# Autodesk Inventor assembly: 69. Блок шестерен промежуточного вала
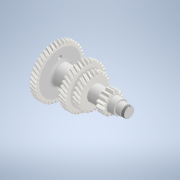
[picture p0: Inventor's stored thumbnail of the model, 180x180]
Saved by Autodesk Inventor 2021 (Build 250183000, 183)
## iProperties
Created: 2021-03-22
Part Number: 69. Блок шестерен промежуточного вала
Document SubType Name: Assembly
Designer: Данил
Author: Данил
## Documents named in this file (6)
- C:\Users\Данил\Desktop\Коробка передач\Детали\69. Блок шестерен промежуточного вала.iam
- C:\Users\Данил\Desktop\Коробка передач\Детали\69. Блок шестерен промежуточного вала.ipt
- C:\Users\Данил\Desktop\Коробка передач\Детали\69. Блок шестерен промежуточного вала\Мастер проектирования\Цилиндрическое зубчатое зацепление1.iam
- C:\Users\Данил\Desktop\Коробка передач\Детали\69. Блок шестерен промежуточного вала\Мастер проектирования\Цилиндрическое зубчатое зацепление2.iam
- C:\Users\Данил\Desktop\Коробка передач\Детали\69. Блок шестерен промежуточного вала\Мастер проектирования\Цилиндрическое зубчатое зацепление3.iam
- C:\Users\Данил\Desktop\Коробка передач\Детали\69. Блок шестерен промежуточного вала\Мастер проектирования\Цилиндрическое зубчатое зацепление4.iam
## Components (5 placed, 2 different names)
1. 69. Блок шестерен промежуточного вала:1 — Совмещение:1, Заподлицо:1, Совмещение:2, Совмещение:3, Совмещение:4, Совмещение:5, Совмещение:6, Совмещение:7
2. Цилиндрическое зубчатое зацепление:1 [sub-assembly] — Совмещение:1, Заподлицо:1
3. Цилиндрическое зубчатое зацепление:2 [sub-assembly] — Совмещение:2, Совмещение:3
4. Цилиндрическое зубчатое зацепление:3 [sub-assembly] — Совмещение:4, Совмещение:5
5. Цилиндрическое зубчатое зацепление:4 [sub-assembly] — Совмещение:6, Совмещение:7
## Relationships (8: Mate 7, Flush 1)
- Совмещение:1 [Mate]: 69. Блок шестерен промежуточного вала:1 ↔ Цилиндрическое зубчатое зацепление:1
- Заподлицо:1 [Flush]: 69. Блок шестерен промежуточного вала:1 ↔ Цилиндрическое зубчатое зацепление:1
- Совмещение:2 [Mate]: 69. Блок шестерен промежуточного вала:1 ↔ Цилиндрическое зубчатое зацепление:2
- Совмещение:3 [Mate]: 69. Блок шестерен промежуточного вала:1 ↔ Цилиндрическое зубчатое зацепление:2
- Совмещение:4 [Mate]: 69. Блок шестерен промежуточного вала:1 ↔ Цилиндрическое зубчатое зацепление:3
- Совмещение:5 [Mate]: 69. Блок шестерен промежуточного вала:1 ↔ Цилиндрическое зубчатое зацепление:3
- Совмещение:6 [Mate]: 69. Блок шестерен промежуточного вала:1 ↔ Цилиндрическое зубчатое зацепление:4
- Совмещение:7 [Mate]: 69. Блок шестерен промежуточного вала:1 ↔ Цилиндрическое зубчатое зацепление:4
